# Autodesk Inventor assembly: turret_assembly
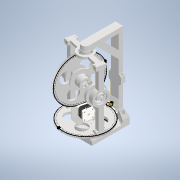
[picture p0: Inventor's stored thumbnail of the model, 180x180]
Saved by Autodesk Inventor 2021 (Build 250183000, 183)
## iProperties
Created: 2020-09-03
Part Number: turret_assembly
Document SubType Name: Assembly
Designer: bober
Author: bober
## Documents named in this file (15)
- D:\Turret\Models\turret_assembly.iam
- D:\Turret\Models\turret_assembly\Design Accelerator\vertical_axis_small_gear.ipt
- D:\Turret\Models\turret_assembly\Design Accelerator\vertical_axis_bigl_gear.ipt
- D:\Turret\Models\turret_assembly\Design Accelerator\horizontal_axis_big_gear.ipt
- D:\Turret\Models\turret_assembly\Design Accelerator\pylon.ipt
- D:\Turret\Models\turret_assembly\Design Accelerator\upper_grip.ipt
- D:\Turret\Models\turret_assembly\Design Accelerator\main_stand_lower_half.ipt
- D:\Turret\Models\turret_assembly\Design Accelerator\main_stand_upper_half.ipt
- D:\Turret\Models\step_motor\Nema 17 Motor a Pasos 17HS4401.iam
- D:\Turret\Models\turret_assembly\Design Accelerator\horizontal_lower_bearing_holder.ipt
- D:\Turret\Models\turret_assembly\Design Accelerator\horizontal_axis_motor_metal_holder.ipt
- D:\Turret\Models\turret_assembly\Design Accelerator\vertical_axis_motor_metal_holder.ipt
- D:\Turret\Models\turret_assembly\Design Accelerator\Swash_distance.ipt
- D:\Turret\Models\turret_assembly\Design Accelerator\small_actuator_holder.ipt
- D:\Turret\Models\turret_assembly\Design Accelerator\big_actuator_holder.ipt
## Components (18 placed, 14 different names)
1. vertical_axis_small_gear:1 — Rigid:4
2. horizontal_axis_big_gear:1 — Rigid:18, Rigid:19
3. vertical_axis_small_gear:2 — Rotational:14
4. vertical_axis_bigl_gear:2 — Rigid:11, Rigid:12, Rigid:20, Rigid:21
5. pylon:1 — Rigid:21
6. pylon:2 — Rigid:20, Rigid:22
7. upper_grip:1 — Rigid:22
8. main_stand_lower_half:1 — Rigid:5, Rotational:12, Mate:1, Mate:2, Rigid:15
9. main_stand_upper_half:1 — Rigid:15
10. Nema 17 Motor a Pasos 17HS4401:2 [sub-assembly] — Rigid:4, Rigid:16
11. Nema 17 Motor a Pasos 17HS4401:3 [sub-assembly] — Rigid:13, Rotational:14
12. horizontal_lower_bearing_holder:1 — Rigid:11, Rotational:11
13. horizontal_axis_motor_metal_holder:1 — Rigid:12, Rigid:13
14. vertical_axis_motor_metal_holder:1 — Rigid:5, Rigid:16
15. Swash_distance:1 — Rotational:11, Rotational:12
16. small_actuator_holder:1 — Rotational:15
17. small_actuator_holder:2 — Rigid:18
18. big_actuator_holder:1 — Rigid:19, Rotational:15
## Relationships (18: WeldJoint 12, RevoluteJoint 4, Mate 2)
- Rigid:4 [WeldJoint]: vertical_axis_small_gear:1 ↔ Nema 17 Motor a Pasos 17HS4401:2
- Rigid:5 [WeldJoint]: main_stand_lower_half:1 ↔ vertical_axis_motor_metal_holder:1
- Rigid:11 [WeldJoint]: vertical_axis_bigl_gear:2 ↔ horizontal_lower_bearing_holder:1
- Rotational:11 [RevoluteJoint]: horizontal_lower_bearing_holder:1 ↔ Swash_distance:1
- Rotational:12 [RevoluteJoint]: main_stand_lower_half:1 ↔ Swash_distance:1
- Mate:1: main_stand_lower_half:1
- Mate:2: main_stand_lower_half:1
- Rigid:12 [WeldJoint]: vertical_axis_bigl_gear:2 ↔ horizontal_axis_motor_metal_holder:1
- Rigid:13 [WeldJoint]: Nema 17 Motor a Pasos 17HS4401:3 ↔ horizontal_axis_motor_metal_holder:1
- Rotational:14 [RevoluteJoint]: vertical_axis_small_gear:2 ↔ Nema 17 Motor a Pasos 17HS4401:3
- Rigid:15 [WeldJoint]: main_stand_lower_half:1 ↔ main_stand_upper_half:1
- Rigid:16 [WeldJoint]: Nema 17 Motor a Pasos 17HS4401:2 ↔ vertical_axis_motor_metal_holder:1
- Rigid:18 [WeldJoint] (-51.5 mm): horizontal_axis_big_gear:1 ↔ small_actuator_holder:2
- Rigid:19 [WeldJoint]: horizontal_axis_big_gear:1 ↔ big_actuator_holder:1
- Rigid:20 [WeldJoint]: vertical_axis_bigl_gear:2 ↔ pylon:2
- Rigid:21 [WeldJoint]: vertical_axis_bigl_gear:2 ↔ pylon:1
- Rigid:22 [WeldJoint]: pylon:2 ↔ upper_grip:1
- Rotational:15 [RevoluteJoint] (55.5 mm): small_actuator_holder:1 ↔ big_actuator_holder:1
